# Autodesk Inventor assembly: CH3-chassisFull
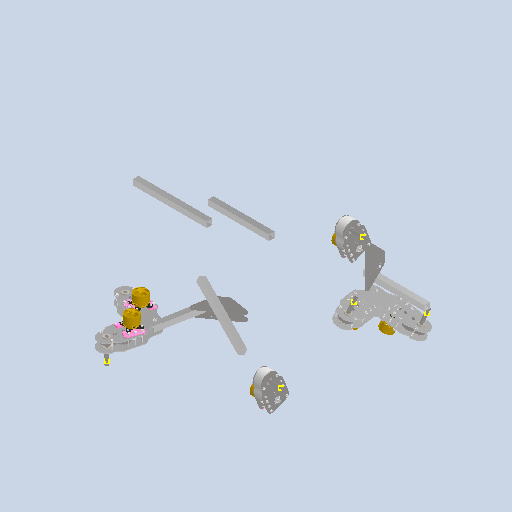
[picture p0: Inventor's stored thumbnail of the model, 512x512]
Saved by Autodesk Inventor 2025.1 (Build 291241020, 241B)
## iProperties
Created: 2025-01-30
Part Number: CH3-chassisFull
Document SubType Name: Assembly
Designer: t205b
Author: t205b
## Documents named in this file (11)
- C:\Users\t205b\OneDrive\Documents\Github\BehrendURCMechanical\CAD\Chassis V3\CH3-chassisFull.iam
- C:\Users\t205b\OneDrive\Documents\Github\BehrendURCMechanical\CAD\Chassis V3\aluminumextrusiontool.ipt
- C:\Users\t205b\OneDrive\Documents\Github\BehrendURCMechanical\CAD\Chassis V3\CH3-L3DoubleGearbox.iam
- C:\Users\t205b\OneDrive\Documents\Github\BehrendURCMechanical\CAD\Chassis V3\CH3-L1SingleGearbox.iam
- C:\Users\t205b\OneDrive\Documents\Github\BehrendURCMechanical\CAD\Chassis V3\HipPivotPlate.ipt
- C:\Users\t205b\OneDrive\Documents\Github\BehrendURCMechanical\CAD\Chassis V3\CH3-PivotBoltNutWasher.iam
- C:\Users\t205b\OneDrive\Documents\Github\BehrendURCMechanical\CAD\Chassis V3\aluminumextrusiontool\aluminumextrusiontool-13.31255in.ipt
- C:\Users\t205b\OneDrive\Documents\Github\BehrendURCMechanical\CAD\Chassis V3\aluminumextrusiontool\aluminumextrusiontool\aluminumextrusiontool-17-13.31255in.ipt
- C:\Users\t205b\OneDrive\Documents\Github\BehrendURCMechanical\CAD\Chassis V3\aluminumextrusiontool\aluminumextrusiontool.ipt
- C:\Users\t205b\OneDrive\Documents\Github\BehrendURCMechanical\CAD\Chassis V3\aluminumextrusiontool\aluminumextrusiontool\aluminumextrusiontool-8in.ipt
- C:\Users\t205b\OneDrive\Documents\Github\BehrendURCMechanical\CAD\Chassis V3\aluminumextrusiontool\aluminumextrusiontool\aluminumextrusiontool-11in.ipt
## Components (14 placed, 8 different names)
1. aluminumextrusiontool-17-13.31255in:11
2. aluminumextrusiontool-8in:12 — Mate:9, Mate:10, Mate:15
3. CH3-L3DoubleGearbox:1 [sub-assembly] — Mate:1, Mate:2
4. CH3-L3DoubleGearbox:2 [sub-assembly] — Mate:4, Mate:5
5. CH3-L1SingleGearbox:1 [sub-assembly]
6. CH3-L1SingleGearbox:2 [sub-assembly]
7. HipPivotPlate:1 — Mate:10
8. HipPivotPlate:2
9. CH3-PivotBoltNutWasher:1 [sub-assembly] — Mate:1, Mate:2, Mate:9
10. CH3-PivotBoltNutWasher:2 [sub-assembly] — Mate:4, Mate:5
11. HipPivotPlate:3 — Mate:15
12. aluminumextrusiontool-11in:13
13. aluminumextrusiontool-11in:14
14. aluminumextrusiontool-13.31255in:10
## Relationships (7: Mate 7)
- Mate:1: CH3-L3DoubleGearbox:1 ↔ CH3-PivotBoltNutWasher:1
- Mate:2: CH3-L3DoubleGearbox:1 ↔ CH3-PivotBoltNutWasher:1
- Mate:4: CH3-L3DoubleGearbox:2 ↔ CH3-PivotBoltNutWasher:2
- Mate:5: CH3-L3DoubleGearbox:2 ↔ CH3-PivotBoltNutWasher:2
- Mate:9: aluminumextrusiontool-8in:12 ↔ CH3-PivotBoltNutWasher:1
- Mate:10: aluminumextrusiontool-8in:12 ↔ HipPivotPlate:1
- Mate:15: aluminumextrusiontool-8in:12 ↔ HipPivotPlate:3
